# Autodesk Inventor assembly: main gripper assembly
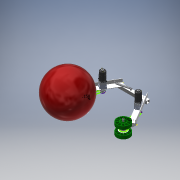
[picture p0: Inventor's stored thumbnail of the model, 180x180]
Saved by Autodesk Inventor 2018 (Build 220112000, 112)
## iProperties
Created: 2019-02-23
Part Number: main gripper assembly
Document SubType Name: Assembly
Designer: s-2513225
Author: s-2513225
## Documents named in this file (16)
- H:\GitHub\2019CAD\NEW NEW GRIPPER (feb 23)\main gripper assembly.iam
- H:\GitHub\2019CAD\NEW NEW GRIPPER (feb 23)\wheel tip connector 1.ipt
- H:\GitHub\2019CAD\NEW NEW GRIPPER (feb 23)\angle iron with  holes 2.ipt
- H:\GitHub\2019CAD\NEW NEW GRIPPER (feb 23)\base mount.ipt
- H:\GitHub\2019CAD\NEW NEW GRIPPER (feb 23)\wheel tip assembly 2018 ver.iam
- H:\GitHub\2019CAD\NEW NEW GRIPPER (feb 23)\wheel tip connector 1_MIR.ipt
- H:\GitHub\2019CAD\NEW NEW GRIPPER (feb 23)\angle iron with  holes 2_MIR.ipt
- H:\GitHub\2019CAD\NEW NEW GRIPPER (feb 23)\wheel tip assembly 2018 ver_MIR.iam
- H:\GitHub\2019CAD\NEW NEW GRIPPER (feb 23)\motor assembly_MIR.iam
- H:\GitHub\2019CAD\NEW NEW GRIPPER (feb 23)\motor assembly_MIR_MIR.iam
- H:\GitHub\2019CAD\NEW NEW GRIPPER (feb 23)\wheel tip connector 1_MIR_MIR.ipt
- H:\GitHub\2019CAD\NEW NEW GRIPPER (feb 23)\angle iron with  holes 2_MIR_MIR.ipt
- H:\GitHub\2019CAD\NEW NEW GRIPPER (feb 23)\wheel tip assembly 2018 ver_MIR_MIR.iam
- H:\GitHub\2019CAD\NEW NEW GRIPPER (feb 23)\ball dummy.ipt
- H:\GitHub\2019CAD\NEW NEW GRIPPER (feb 23)\eye screw stand-in.ipt
- H:\GitHub\2019CAD\NEW NEW GRIPPER (feb 23)\spring stand in.ipt
## Components (16 placed, 15 different names)
1. wheel tip connector 1:1 — Mate:12, Mate:23, Mate:25
2. angle iron with  holes 2:1 — Mate:12, Mate:14, Mate:19, Mate:20, Mate:21, Mate:24
3. base mount:1 — Mate:14, Mate:19, Mate:26, Mate:34, Mate:35, Mate:42, Mate:43, Mate:44, Mate:51, Flush:2
4. wheel tip assembly 2018 ver:1 [sub-assembly] — Mate:20, Mate:21, Mate:23, Mate:24, Mate:25
5. wheel tip connector 1_MIR:1 — Mate:28, Mate:29, Mate:31, Mate:49
6. angle iron with  holes 2_MIR:1 — Mate:28, Mate:30, Mate:32, Mate:34, Mate:35, Mate:47, Mate:48, Mate:49, Mate:50, Mate:52
7. wheel tip assembly 2018 ver_MIR:1 [sub-assembly] — Mate:29, Mate:30, Mate:31, Mate:32, Mate:50
8. motor assembly_MIR:1 [sub-assembly] — Mate:47, Mate:48
9. motor assembly_MIR_MIR:1 [sub-assembly] — Mate:45, Mate:46
10. wheel tip connector 1_MIR_MIR:1 — Mate:36, Mate:39, Mate:41
11. angle iron with  holes 2_MIR_MIR:1 — Mate:36, Mate:37, Mate:38, Mate:40, Mate:42, Mate:43, Mate:44, Mate:45, Mate:46
12. wheel tip assembly 2018 ver_MIR_MIR:1 [sub-assembly] — Mate:37, Mate:38, Mate:39, Mate:40, Mate:41
13. ball dummy:1
14. eye screw stand-in:1 — Mate:52
15. eye screw stand-in:2 — Mate:51, Flush:2
16. spring stand in:1
## Relationships (35: Mate 33, Flush 2)
- Mate:12: wheel tip connector 1:1 ↔ angle iron with  holes 2:1
- Mate:14: angle iron with  holes 2:1 ↔ base mount:1
- Mate:19: angle iron with  holes 2:1 ↔ base mount:1
- Mate:20: angle iron with  holes 2:1 ↔ wheel tip assembly 2018 ver:1
- Mate:21: angle iron with  holes 2:1 ↔ wheel tip assembly 2018 ver:1
- Mate:23: wheel tip connector 1:1 ↔ wheel tip assembly 2018 ver:1
- Mate:24: angle iron with  holes 2:1 ↔ wheel tip assembly 2018 ver:1
- Mate:25: wheel tip connector 1:1 ↔ wheel tip assembly 2018 ver:1
- Mate:26: base mount:1
- Flush:1 (63.5 mm)
- Mate:28: wheel tip connector 1_MIR:1 ↔ angle iron with  holes 2_MIR:1
- Mate:29: wheel tip connector 1_MIR:1 ↔ wheel tip assembly 2018 ver_MIR:1
- Mate:30: angle iron with  holes 2_MIR:1 ↔ wheel tip assembly 2018 ver_MIR:1
- Mate:31: wheel tip connector 1_MIR:1 ↔ wheel tip assembly 2018 ver_MIR:1
- Mate:32: angle iron with  holes 2_MIR:1 ↔ wheel tip assembly 2018 ver_MIR:1
- Mate:34: base mount:1 ↔ angle iron with  holes 2_MIR:1
- Mate:35: base mount:1 ↔ angle iron with  holes 2_MIR:1
- Mate:36: wheel tip connector 1_MIR_MIR:1 ↔ angle iron with  holes 2_MIR_MIR:1
- Mate:37: angle iron with  holes 2_MIR_MIR:1 ↔ wheel tip assembly 2018 ver_MIR_MIR:1
- Mate:38: angle iron with  holes 2_MIR_MIR:1 ↔ wheel tip assembly 2018 ver_MIR_MIR:1
- Mate:39: wheel tip connector 1_MIR_MIR:1 ↔ wheel tip assembly 2018 ver_MIR_MIR:1
- Mate:40: angle iron with  holes 2_MIR_MIR:1 ↔ wheel tip assembly 2018 ver_MIR_MIR:1
- Mate:41: wheel tip connector 1_MIR_MIR:1 ↔ wheel tip assembly 2018 ver_MIR_MIR:1
- Mate:42: base mount:1 ↔ angle iron with  holes 2_MIR_MIR:1
- Mate:43: base mount:1 ↔ angle iron with  holes 2_MIR_MIR:1
- Mate:44: base mount:1 ↔ angle iron with  holes 2_MIR_MIR:1
- Mate:45: motor assembly_MIR_MIR:1 ↔ angle iron with  holes 2_MIR_MIR:1
- Mate:46: motor assembly_MIR_MIR:1 ↔ angle iron with  holes 2_MIR_MIR:1
- Mate:47: angle iron with  holes 2_MIR:1 ↔ motor assembly_MIR:1
- Mate:48: angle iron with  holes 2_MIR:1 ↔ motor assembly_MIR:1
- Mate:49: wheel tip connector 1_MIR:1 ↔ angle iron with  holes 2_MIR:1
- Mate:50: angle iron with  holes 2_MIR:1 ↔ wheel tip assembly 2018 ver_MIR:1
- Mate:51 (-18.796 mm): base mount:1 ↔ eye screw stand-in:2
- Flush:2 (114.3 mm): base mount:1 ↔ eye screw stand-in:2
- Mate:52 (-18.796 mm): angle iron with  holes 2_MIR:1 ↔ eye screw stand-in:1
